# Autodesk Inventor assembly: P1704_E001
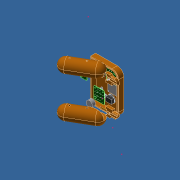
[picture p0: Inventor's stored thumbnail of the model, 180x180]
Saved by Autodesk Inventor 2019 (Build 230136000, 136)
## iProperties
Created: 2019-04-29
Part Number: P1704_E001
Material: Générique
Document SubType Name: Assembly
Designer: Joan.MAILLARD
Author: Joan.MAILLARD
## Documents named in this file (19)
- P:\projet_manette\manette\06_Dessins\2019\Manette universelle\P1704_E001.iam
- P:\projet_manette\manette\06_Dessins\2019\Manette universelle\P1704_004_mainDroiteExterieur.ipt
- P:\projet_manette\manette\06_Dessins\2019\Manette universelle\P1704_005_mainGaucheExterieur.ipt
- P:\projet_manette\manette\06_Dessins\2019\Manette universelle\P1704_001_basManette.ipt
- P:\projet_manette\manette\06_Dessins\2019\Manette universelle\P1704_006_gachette.ipt
- P:\projet_manette\manette\06_Dessins\2019\Manette universelle\P1704_007_guideRessort.ipt
- P:\projet_manette\manette\06_Dessins\2019\Manette universelle\P1704_002_mainDroiteInterieur.ipt
- P:\projet_manette\manette\06_Dessins\2019\Manette universelle\P1704_003_mainGaucheInterieur.ipt
- P:\projet_manette\manette\06_Dessins\2019\Manette universelle\P1704_009_slider.ipt
- P:\projet_manette\manette\06_Dessins\2019\Manette universelle\P1704_011_4buttonPCB.ipt
- P:\projet_manette\manette\06_Dessins\2019\Manette universelle\P1704_010_startSelectPCB.ipt
- P:\projet_manette\manette\06_Dessins\2019\Manette universelle\P1704_012_joystick.ipt
- P:\projet_manette\manette\06_Dessins\2019\Manette universelle\P1704_014_Display.ipt
- P:\projet_manette\manette\06_Dessins\2019\Manette universelle\P1704_015_rumble.ipt
- P:\projet_manette\manette\06_Dessins\2019\Manette universelle\P1704_008_pcb.ipt
- P:\projet_manette\manette\06_Dessins\2019\Manette universelle\P1704_018_hautManette.ipt
- P:\projet_manette\manette\06_Dessins\2019\Manette universelle\P1704_E003_button.iam
- P:\projet_manette\manette\06_Dessins\2019\Manette universelle\P1704_016_Button.ipt
- P:\projet_manette\manette\06_Dessins\2019\Manette universelle\P1704_019_button_triangle_cap.ipt
## Components (33 placed, 18 different names)
1. P1704_004_mainDroiteExterieur:1 — Rotation:7, Rotation:8, Placage:14
2. P1704_005_mainGaucheExterieur:1 — Rotation:9, Rotation:10, Placage:12
3. P1704_001_basManette:1 — Placage:11, Placage:12, Placage:13, Placage:14, Placage:20, Placage:22, Placage:24, Placage:26, Placage:27, Placage:30, Placage:31, Placage:32, Placage:33, Placage:34, Placage:35, Placage:38, Placage:41, Placage:42, Placage:43, Placage:49, Affleurement:4, Affleurement:5
4. P1704_006_gachette:1 — Rotation:2, Glissière:4, Placage:26, Placage:27, Affleurement:1
5. P1704_006_gachette:2 — Rotation:1, Glissière:3
6. P1704_007_guideRessort:1 — Rotation:1
7. P1704_007_guideRessort:2 — Rotation:2
8. P1704_002_mainDroiteInterieur:1 — Rotation:7, Rotation:8, Placage:13
9. P1704_003_mainGaucheInterieur:1 — Rotation:9, Rotation:10, Placage:11
10. P1704_009_slider:1 — Glissière:3
11. P1704_009_slider:2 — Glissière:4, Affleurement:1
12. manette_2019_boutons.kicad_pcb_Contour:1 — Placage:22, Placage:52, Placage:53, Placage:54, Placage:56, Angle:1, Angle:2, Placage:57, Placage:58, Placage:59, Placage:60, Angle:3, Placage:61, Placage:62, Placage:63, Angle:4, Placage:64, Placage:65
13. manette_2019_boutons.kicad_pcb_Contour:2 — Placage:20, Placage:66, Placage:67, Placage:68, Placage:69, Placage:70, Angle:5, Angle:6, Angle:7, Angle:8, Placage:71, Placage:72, Placage:73, Placage:74, Placage:75, Placage:76, Placage:77, Angle:9, Angle:10, Angle:11, Angle:12, Placage:86
14. Manette_2019_PCB_Central.kicad_pcb_Contour:1 — Placage:24, Placage:87
15. P1704_012_joystick:1 — Placage:30, Placage:31, Placage:48
16. P1704_012_joystick:2 — Placage:32, Placage:33, Placage:47
17. P1704_014_Display:1 — Placage:38, Placage:50
18. P1704_015_rumble:1 — Placage:34
19. P1704_015_rumble:2 — Placage:35
20. manette_2019.kicad_pcb_Contour:1 — Placage:41, Placage:42, Placage:43, Placage:47, Placage:48
21. P1704_018_hautManette:1 — Placage:49, Affleurement:4, Affleurement:5, Placage:50, Placage:65, Placage:86, Placage:87
22. P1704_E003_button:1 [sub-assembly] — Placage:56, Angle:2, Placage:57, Placage:58
23. P1704_E003_button:2 [sub-assembly] — Placage:52, Placage:53, Placage:54, Angle:1
24. P1704_E003_button:3 [sub-assembly] — Placage:59, Placage:63, Angle:4, Placage:64
25. P1704_E003_button:4 [sub-assembly] — Placage:60, Angle:3, Placage:61, Placage:62
26. P1704_016_Button:1 — Placage:68, Angle:7, Placage:76, Placage:77, Placage:84, Placage:85
27. P1704_016_Button:2 — Placage:66, Angle:8, Placage:74, Placage:75, Placage:82, Placage:83
28. P1704_016_Button:3 — Placage:69, Angle:6, Placage:72, Placage:73, Placage:80, Placage:81
29. P1704_016_Button:4 — Placage:67, Placage:70, Angle:5, Placage:71, Placage:78, Placage:79
30. P1704_019_button_triangle_cap:1 — Placage:82, Placage:83, Angle:12
31. P1704_019_button_triangle_cap:2 — Placage:84, Placage:85, Angle:11
32. P1704_019_button_triangle_cap:3 — Placage:78, Placage:79, Angle:10
33. P1704_019_button_triangle_cap:4 — Placage:80, Placage:81, Angle:9
## Relationships (81: Mate 58, Angle 12, RevoluteJoint 6, Flush 3, TranslationJoint 2)
- Rotation:1 [RevoluteJoint] (4.5 mm): P1704_006_gachette:2 ↔ P1704_007_guideRessort:1
- Rotation:2 [RevoluteJoint] (4.5 mm): P1704_006_gachette:1 ↔ P1704_007_guideRessort:2
- Rotation:7 [RevoluteJoint]: P1704_004_mainDroiteExterieur:1 ↔ P1704_002_mainDroiteInterieur:1
- Rotation:8 [RevoluteJoint]: P1704_004_mainDroiteExterieur:1 ↔ P1704_002_mainDroiteInterieur:1
- Rotation:9 [RevoluteJoint]: P1704_005_mainGaucheExterieur:1 ↔ P1704_003_mainGaucheInterieur:1
- Rotation:10 [RevoluteJoint]: P1704_005_mainGaucheExterieur:1 ↔ P1704_003_mainGaucheInterieur:1
- Glissière:3 [TranslationJoint]: P1704_006_gachette:2 ↔ P1704_009_slider:1
- Glissière:4 [TranslationJoint]: P1704_006_gachette:1 ↔ P1704_009_slider:2
- Placage:11 [Mate]: P1704_001_basManette:1 ↔ P1704_003_mainGaucheInterieur:1
- Placage:12 [Mate]: P1704_005_mainGaucheExterieur:1 ↔ P1704_001_basManette:1
- Placage:13 [Mate]: P1704_001_basManette:1 ↔ P1704_002_mainDroiteInterieur:1
- Placage:14 [Mate]: P1704_004_mainDroiteExterieur:1 ↔ P1704_001_basManette:1
- Placage:20 [Mate] (10 mm): P1704_001_basManette:1 ↔ manette_2019_boutons.kicad_pcb_Contour:2
- Placage:22 [Mate] (5 mm): P1704_001_basManette:1 ↔ manette_2019_boutons.kicad_pcb_Contour:1
- Placage:24 [Mate] (57.5375 mm): P1704_001_basManette:1 ↔ Manette_2019_PCB_Central.kicad_pcb_Contour:1
- Placage:26 [Mate]: P1704_001_basManette:1 ↔ P1704_006_gachette:1
- Placage:27 [Mate]: P1704_001_basManette:1 ↔ P1704_006_gachette:1
- Affleurement:1 [Flush]: P1704_006_gachette:1 ↔ P1704_009_slider:2
- Placage:30 [Mate] (35 mm): P1704_001_basManette:1 ↔ P1704_012_joystick:1
- Placage:31 [Mate] (40 mm): P1704_001_basManette:1 ↔ P1704_012_joystick:1
- Placage:32 [Mate] (35 mm): P1704_001_basManette:1 ↔ P1704_012_joystick:2
- Placage:33 [Mate] (35 mm): P1704_001_basManette:1 ↔ P1704_012_joystick:2
- Placage:34 [Mate]: P1704_001_basManette:1 ↔ P1704_015_rumble:1
- Placage:35 [Mate]: P1704_001_basManette:1 ↔ P1704_015_rumble:2
- Placage:38 [Mate] (53.375 mm): P1704_001_basManette:1 ↔ P1704_014_Display:1
- Placage:41 [Mate]: P1704_001_basManette:1 ↔ manette_2019.kicad_pcb_Contour:1
- Placage:42 [Mate]: P1704_001_basManette:1 ↔ manette_2019.kicad_pcb_Contour:1
- Placage:43 [Mate]: P1704_001_basManette:1 ↔ manette_2019.kicad_pcb_Contour:1
- Placage:47 [Mate] (7 mm): P1704_012_joystick:2 ↔ manette_2019.kicad_pcb_Contour:1
- Placage:48 [Mate] (7 mm): P1704_012_joystick:1 ↔ manette_2019.kicad_pcb_Contour:1
- Placage:49 [Mate]: P1704_001_basManette:1 ↔ P1704_018_hautManette:1
- Affleurement:4 [Flush]: P1704_001_basManette:1 ↔ P1704_018_hautManette:1
- Affleurement:5 [Flush]: P1704_001_basManette:1 ↔ P1704_018_hautManette:1
- Placage:50 [Mate]: P1704_014_Display:1 ↔ P1704_018_hautManette:1
- Placage:52 [Mate]: manette_2019_boutons.kicad_pcb_Contour:1 ↔ P1704_E003_button:2
- Placage:53 [Mate] (-37.465 mm): manette_2019_boutons.kicad_pcb_Contour:1 ↔ P1704_E003_button:2
- Placage:54 [Mate] (-19.05 mm): manette_2019_boutons.kicad_pcb_Contour:1 ↔ P1704_E003_button:2
- Placage:56 [Mate] (-24.765 mm): manette_2019_boutons.kicad_pcb_Contour:1 ↔ P1704_E003_button:1
- Angle:1 (0 deg): manette_2019_boutons.kicad_pcb_Contour:1 ↔ P1704_E003_button:2
- Angle:2 (0 deg): manette_2019_boutons.kicad_pcb_Contour:1 ↔ P1704_E003_button:1
- Placage:57 [Mate]: manette_2019_boutons.kicad_pcb_Contour:1 ↔ P1704_E003_button:1
- Placage:58 [Mate] (-30.48 mm): manette_2019_boutons.kicad_pcb_Contour:1 ↔ P1704_E003_button:1
- Placage:59 [Mate]: manette_2019_boutons.kicad_pcb_Contour:1 ↔ P1704_E003_button:3
- Placage:60 [Mate]: manette_2019_boutons.kicad_pcb_Contour:1 ↔ P1704_E003_button:4
- Angle:3 (0 deg): manette_2019_boutons.kicad_pcb_Contour:1 ↔ P1704_E003_button:4
- Placage:61 [Mate] (-24.765 mm): manette_2019_boutons.kicad_pcb_Contour:1 ↔ P1704_E003_button:4
- Placage:62 [Mate] (-7.62 mm): manette_2019_boutons.kicad_pcb_Contour:1 ↔ P1704_E003_button:4
- Placage:63 [Mate] (-12.065 mm): manette_2019_boutons.kicad_pcb_Contour:1 ↔ P1704_E003_button:3
- Angle:4 (0 deg): manette_2019_boutons.kicad_pcb_Contour:1 ↔ P1704_E003_button:3
- Placage:64 [Mate] (-19.05 mm): manette_2019_boutons.kicad_pcb_Contour:1 ↔ P1704_E003_button:3
- Placage:65 [Mate] (10 mm): manette_2019_boutons.kicad_pcb_Contour:1 ↔ P1704_018_hautManette:1
- Placage:66 [Mate]: manette_2019_boutons.kicad_pcb_Contour:2 ↔ P1704_016_Button:2
- Placage:67 [Mate]: manette_2019_boutons.kicad_pcb_Contour:2 ↔ P1704_016_Button:4
- Placage:68 [Mate]: manette_2019_boutons.kicad_pcb_Contour:2 ↔ P1704_016_Button:1
- Placage:69 [Mate]: manette_2019_boutons.kicad_pcb_Contour:2 ↔ P1704_016_Button:3
- Placage:70 [Mate] (-7.62 mm): manette_2019_boutons.kicad_pcb_Contour:2 ↔ P1704_016_Button:4
- Angle:5 (0 deg): manette_2019_boutons.kicad_pcb_Contour:2 ↔ P1704_016_Button:4
- Angle:6 (0 deg): manette_2019_boutons.kicad_pcb_Contour:2 ↔ P1704_016_Button:3
- Angle:7 (0 deg): manette_2019_boutons.kicad_pcb_Contour:2 ↔ P1704_016_Button:1
- Angle:8 (0 deg): manette_2019_boutons.kicad_pcb_Contour:2 ↔ P1704_016_Button:2
- Placage:71 [Mate] (-24.765 mm): manette_2019_boutons.kicad_pcb_Contour:2 ↔ P1704_016_Button:4
- Placage:72 [Mate] (-12.065 mm): manette_2019_boutons.kicad_pcb_Contour:2 ↔ P1704_016_Button:3
- Placage:73 [Mate] (-19.05 mm): manette_2019_boutons.kicad_pcb_Contour:2 ↔ P1704_016_Button:3
- Placage:74 [Mate] (-30.48 mm): manette_2019_boutons.kicad_pcb_Contour:2 ↔ P1704_016_Button:2
- Placage:75 [Mate] (-24.765 mm): manette_2019_boutons.kicad_pcb_Contour:2 ↔ P1704_016_Button:2
- Placage:76 [Mate] (-37.465 mm): manette_2019_boutons.kicad_pcb_Contour:2 ↔ P1704_016_Button:1
- Placage:77 [Mate] (-19.05 mm): manette_2019_boutons.kicad_pcb_Contour:2 ↔ P1704_016_Button:1
- Placage:78 [Mate]: P1704_016_Button:4 ↔ P1704_019_button_triangle_cap:3
- Placage:79 [Mate]: P1704_016_Button:4 ↔ P1704_019_button_triangle_cap:3
- Placage:80 [Mate]: P1704_016_Button:3 ↔ P1704_019_button_triangle_cap:4
- Placage:81 [Mate]: P1704_016_Button:3 ↔ P1704_019_button_triangle_cap:4
- Placage:82 [Mate]: P1704_016_Button:2 ↔ P1704_019_button_triangle_cap:1
- Placage:83 [Mate]: P1704_016_Button:2 ↔ P1704_019_button_triangle_cap:1
- Placage:84 [Mate]: P1704_016_Button:1 ↔ P1704_019_button_triangle_cap:2
- Placage:85 [Mate]: P1704_016_Button:1 ↔ P1704_019_button_triangle_cap:2
- Angle:9 (180 deg): manette_2019_boutons.kicad_pcb_Contour:2 ↔ P1704_019_button_triangle_cap:4
- Angle:10 (180 deg): manette_2019_boutons.kicad_pcb_Contour:2 ↔ P1704_019_button_triangle_cap:3
- Angle:11 (180 deg): manette_2019_boutons.kicad_pcb_Contour:2 ↔ P1704_019_button_triangle_cap:2
- Angle:12 (180 deg): manette_2019_boutons.kicad_pcb_Contour:2 ↔ P1704_019_button_triangle_cap:1
- Placage:86 [Mate] (10 mm): manette_2019_boutons.kicad_pcb_Contour:2 ↔ P1704_018_hautManette:1
- Placage:87 [Mate] (10 mm): Manette_2019_PCB_Central.kicad_pcb_Contour:1 ↔ P1704_018_hautManette:1
